# Autodesk Inventor assembly: clamp_
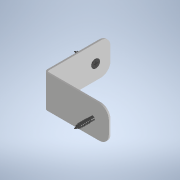
[picture p0: Inventor's stored thumbnail of the model, 180x180]
Saved by Autodesk Inventor 2021 (Build 250183000, 183)
## iProperties
Created: 2021-07-10
Part Number: clamp_
Document SubType Name: Assembly
Designer: TARUN
Author: TARUN
## Documents named in this file (3)
- G:\Exploration\Team8_new\clamp_.iam
- G:\Exploration\Team8_new\clamp.ipt
- G:\Exploration\Team8_new\screws.ipt
## Components (3 placed, 2 different names)
1. clamp:1 — Mate:1, Flush:1, Mate:2, Flush:2
2. screws:1 — Mate:2, Flush:2
3. screws:2 — Mate:1, Flush:1
## Relationships (4: Mate 2, Flush 2)
- Mate:1: clamp:1 ↔ screws:2
- Flush:1 (-0.5 mm): clamp:1 ↔ screws:2
- Mate:2: clamp:1 ↔ screws:1
- Flush:2 (-0.5 mm): clamp:1 ↔ screws:1
